# Autodesk Inventor assembly: headstage+flex connector_CPY
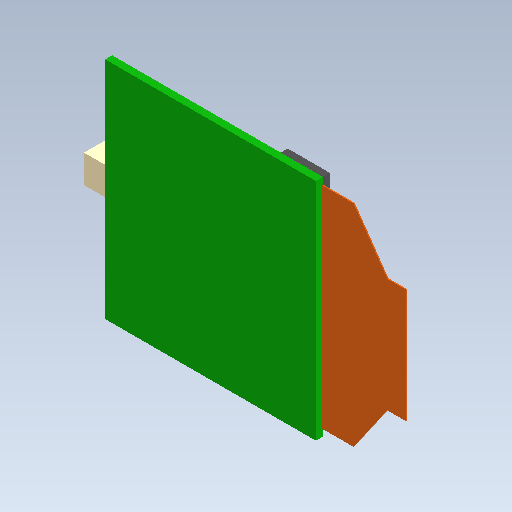
[picture p0: Inventor's stored thumbnail of the model, 512x512]
Saved by Autodesk Inventor 2020 (Build 240168000, 168)
## iProperties
Created: 2020-03-27
Part Number: headstage+flex connector_CPY
Document SubType Name: Assembly
Designer: brodylab
Author: Thomas Zhihao Luo
## Documents named in this file (3)
- C:\Users\brodylab\Desktop\2.611\headstage+flex connector_CPY.iam
- C:\Users\brodylab\Desktop\2.611\headstage_CPY.ipt
- C:\Users\brodylab\Desktop\2.611\flexcable3_CPY.ipt
## Components (2 placed, 2 different names)
1. headstage_CPY:1 — Rigid:1
2. flexcable3_CPY:1 — Rigid:1
## Relationships (1: WeldJoint 1)
- Rigid:1 [WeldJoint]: headstage_CPY:1 ↔ flexcable3_CPY:1
